# Autodesk Inventor assembly: Modulo Sistema Embebido
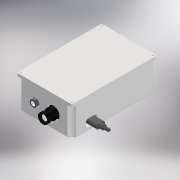
[picture p0: Inventor's stored thumbnail of the model, 180x180]
Saved by Autodesk Inventor 2021.4 (Build 254397000, 397)
## iProperties
Created: 2022-12-12
Part Number: Modulo Sistema Embebido
Document SubType Name: Assembly
Designer: crist
Mass: 674.638 g
Surface Area: 1430.38 cm^2
Volume: 126.282 cm^3
Density: 5.34231 g/cm^3
Author: crist
## Documents named in this file (7)
- C:\Users\crist\OneDrive - Escuela Superior Politécnica del Litoral\Escritorio\Archivos\Dron\Modulo Sistema Embebido.iam
- C:\Users\crist\OneDrive - Escuela Superior Politécnica del Litoral\Escritorio\Archivos\Dron\Raspberry Pi\Chasis Raspberry Pi.ipt
- C:\Users\crist\OneDrive - Escuela Superior Politécnica del Litoral\Escritorio\Archivos\Dron\Raspberry Pi\sistema embebido final.iam
- C:\Users\crist\OneDrive - Escuela Superior Politécnica del Litoral\Escritorio\Archivos\Dron\Raspberry Pi\Raspberry Pi Camera (B) Rev 2.0.iam
- C:\Users\crist\OneDrive - Escuela Superior Politécnica del Litoral\Escritorio\Archivos\Dron\Raspberry Pi\MLX90640.ipt
- C:\Users\crist\OneDrive - Escuela Superior Politécnica del Litoral\Escritorio\Archivos\Dron\Raspberry Pi\Chasis Tapa Raspberry Pi.ipt
- C:\Users\crist\OneDrive - Escuela Superior Politécnica del Litoral\Escritorio\Archivos\Dron\Tornillo 1.ipt
## Components (11 placed, 6 different names)
1. Chasis Raspberry Pi:1 — Rígido:2, Rígido:3, Rígido:4, Rígido:5
2. sistema embebido final:1 [sub-assembly] — Rígido:4
3. Raspberry Pi Camera (B) Rev 2.0:1 [sub-assembly] — Rígido:2, Cilíndrica:1, Cilíndrica:2, Cilíndrica:5, Cilíndrica:6
4. MLX90640:1 — Rígido:3, Cilíndrica:3, Cilíndrica:4
5. Chasis Tapa Raspberry Pi:1 — Rígido:5
6. Tornillo 1:1 — Cilíndrica:1
7. Tornillo 1:2 — Cilíndrica:2
8. Tornillo 1:3 — Cilíndrica:3
9. Tornillo 1:4 — Cilíndrica:4
10. Tornillo 1:5 — Cilíndrica:6
11. Tornillo 1:6 — Cilíndrica:5
## Relationships (10: CylindricalJoint 6, WeldJoint 4)
- Rígido:2 [WeldJoint]: Chasis Raspberry Pi:1 ↔ Raspberry Pi Camera (B) Rev 2.0:1
- Rígido:3 [WeldJoint]: Chasis Raspberry Pi:1 ↔ MLX90640:1
- Rígido:4 [WeldJoint]: Chasis Raspberry Pi:1 ↔ sistema embebido final:1
- Rígido:5 [WeldJoint]: Chasis Raspberry Pi:1 ↔ Chasis Tapa Raspberry Pi:1
- Cilíndrica:1 [CylindricalJoint]: Raspberry Pi Camera (B) Rev 2.0:1 ↔ Tornillo 1:1
- Cilíndrica:2 [CylindricalJoint]: Raspberry Pi Camera (B) Rev 2.0:1 ↔ Tornillo 1:2
- Cilíndrica:3 [CylindricalJoint]: MLX90640:1 ↔ Tornillo 1:3
- Cilíndrica:4 [CylindricalJoint]: MLX90640:1 ↔ Tornillo 1:4
- Cilíndrica:5 [CylindricalJoint]: Raspberry Pi Camera (B) Rev 2.0:1 ↔ Tornillo 1:6
- Cilíndrica:6 [CylindricalJoint]: Raspberry Pi Camera (B) Rev 2.0:1 ↔ Tornillo 1:5
